# Autodesk Inventor assembly: Rod下
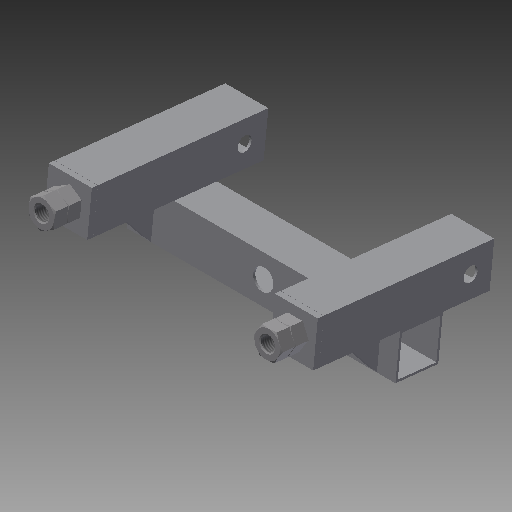
[picture p0: Inventor's stored thumbnail of the model, 512x512]
Saved by Autodesk Inventor 2018 (Build 220112000, 112)
## iProperties
Created: 2017-09-13
Part Number: Rod下
Material: 一般
Document SubType Name: Assembly
Designer: mura5
Author: mura5
## Documents named in this file (6)
- D:\Works\RBBR\cart\前足改\Aアーム下.iam
- D:\Works\RBBR\cart\前足改\PipeB穴あり.ipt
- D:\Works\RBBR\cart\前足改\PipeB蓋.ipt
- D:\Works\RBBR\cart\前足改\hn1_12.ipt
- D:\Works\RBBR\cart\前足改\Pipe横_前.ipt
- D:\Works\RBBR\cart\前足改\リブ.ipt
## Components (11 placed, 5 different names)
1. PipeB穴あり:1 — リジッド:10, メイト:2, フラッシュ:3, メイト:5
2. PipeB蓋:1 — リジッド:2, リジッド:10, フラッシュ:6
3. hn1_12:1 — リジッド:2, リジッド:3
4. hn1_12:2 — リジッド:3
5. Pipe横_前:1 — フラッシュ:1, メイト:1, メイト:2, フラッシュ:3, フラッシュ:5, フラッシュ:6, メイト:4, フラッシュ:7, メイト:6, フラッシュ:8
6. PipeB穴あり:2 — リジッド:9, フラッシュ:1, メイト:1, メイト:3
7. PipeB蓋:2 — リジッド:7, リジッド:9, フラッシュ:5
8. hn1_12:3 — リジッド:7, リジッド:8
9. hn1_12:4 — リジッド:8
10. リブ:1 — メイト:3, メイト:4, フラッシュ:7
11. リブ:2 — メイト:5, メイト:6, フラッシュ:8
## Relationships (18: WeldJoint 6, Flush 6, Mate 6)
- リジッド:2 [WeldJoint]: PipeB蓋:1 ↔ hn1_12:1
- リジッド:3 [WeldJoint]: hn1_12:1 ↔ hn1_12:2
- リジッド:7 [WeldJoint]: PipeB蓋:2 ↔ hn1_12:3
- リジッド:8 [WeldJoint]: hn1_12:3 ↔ hn1_12:4
- リジッド:9 [WeldJoint]: PipeB穴あり:2 ↔ PipeB蓋:2
- リジッド:10 [WeldJoint]: PipeB穴あり:1 ↔ PipeB蓋:1
- フラッシュ:1 [Flush]: Pipe横_前:1 ↔ PipeB穴あり:2
- メイト:1 [Mate]: Pipe横_前:1 ↔ PipeB穴あり:2
- メイト:2 [Mate]: PipeB穴あり:1 ↔ Pipe横_前:1
- フラッシュ:3 [Flush]: PipeB穴あり:1 ↔ Pipe横_前:1
- フラッシュ:5 [Flush] (65 mm): Pipe横_前:1 ↔ PipeB蓋:2
- フラッシュ:6 [Flush] (65 mm): PipeB蓋:1 ↔ Pipe横_前:1
- メイト:3 [Mate]: PipeB穴あり:2 ↔ リブ:1
- メイト:4 [Mate]: Pipe横_前:1 ↔ リブ:1
- フラッシュ:7 [Flush] (13.75 mm): Pipe横_前:1 ↔ リブ:1
- メイト:5 [Mate]: PipeB穴あり:1 ↔ リブ:2
- メイト:6 [Mate]: Pipe横_前:1 ↔ リブ:2
- フラッシュ:8 [Flush] (13.75 mm): Pipe横_前:1 ↔ リブ:2
